# Autodesk Inventor assembly: Top_Rail_Section
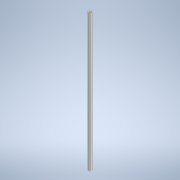
[picture p0: Inventor's stored thumbnail of the model, 180x180]
Saved by Autodesk Inventor 2022 (Build 260153000, 153)
## iProperties
Created: 2021-06-14
Part Number: Top_Rail_Section
Document SubType Name: Assembly
Designer: Jorian Brusind
Author: Jorian Brusind
## Documents named in this file (3)
- C:\Users\Jorian Brusind\Documents\GitHub\HyperRail\Inventor Files\Top_Rail_Section.iam
- C:\Users\Jorian Brusind\Documents\GitHub\HyperRail\Inventor Files\5537T425_T-SLOTTED FRAMING.ipt
- C:\Users\Jorian Brusind\Documents\GitHub\HyperRail\Inventor Files\8020_Sets\IPT_20_Series\IPT_20_Series\20-4040_2m.ipt
## Components (5 placed, 2 different names)
1. 5537T425_T-SLOTTED FRAMING:1 — Mate:7, Mate:8, Mate:9
2. 5537T425_T-SLOTTED FRAMING:2 — Mate:1, Mate:2, Mate:3
3. 5537T425_T-SLOTTED FRAMING:3 — Mate:4, Mate:5, Mate:6
4. 5537T425_T-SLOTTED FRAMING:4 — Mate:10, Mate:11, Mate:12
5. 20-4040_2m:1 — Mate:1, Mate:2, Mate:3, Mate:4, Mate:5, Mate:6, Mate:7, Mate:8, Mate:9, Mate:10, Mate:11, Mate:12
## Relationships (12: Mate 12)
- Mate:1 (1 mm): 5537T425_T-SLOTTED FRAMING:2 ↔ 20-4040_2m:1
- Mate:2: 5537T425_T-SLOTTED FRAMING:2 ↔ 20-4040_2m:1
- Mate:3 (-15 mm): 5537T425_T-SLOTTED FRAMING:2 ↔ 20-4040_2m:1
- Mate:4 (-1 mm): 5537T425_T-SLOTTED FRAMING:3 ↔ 20-4040_2m:1
- Mate:5: 5537T425_T-SLOTTED FRAMING:3 ↔ 20-4040_2m:1
- Mate:6: 5537T425_T-SLOTTED FRAMING:3 ↔ 20-4040_2m:1
- Mate:7: 5537T425_T-SLOTTED FRAMING:1 ↔ 20-4040_2m:1
- Mate:8: 5537T425_T-SLOTTED FRAMING:1 ↔ 20-4040_2m:1
- Mate:9 (-15 mm): 5537T425_T-SLOTTED FRAMING:1 ↔ 20-4040_2m:1
- Mate:10: 5537T425_T-SLOTTED FRAMING:4 ↔ 20-4040_2m:1
- Mate:11: 5537T425_T-SLOTTED FRAMING:4 ↔ 20-4040_2m:1
- Mate:12: 5537T425_T-SLOTTED FRAMING:4 ↔ 20-4040_2m:1
